# Autodesk Inventor assembly: Assembly1 DOLORIMETRO FINAL (ESPERO)
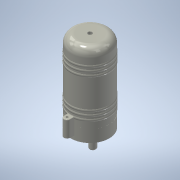
[picture p0: Inventor's stored thumbnail of the model, 180x180]
Saved by Autodesk Inventor 2022 (Build 260153000, 153)
## iProperties
Created: 2022-11-21
Part Number: Assembly1 DOLORIMETRO FINAL (ESPERO)
Document SubType Name: Assembly
Designer: ASUS
Author: ASUS
## Documents named in this file (5)
- C:\CICLO IV\FUNDAMENTOS DE BIODISEÑO\BIODEÑO\Assembly1 DOLORIMETRO FINAL (ESPERO).iam
- C:\CICLO IV\FUNDAMENTOS DE BIODISEÑO\BIODEÑO\BARRA V3 (1).ipt
- C:\CICLO IV\FUNDAMENTOS DE BIODISEÑO\BIODEÑO\Carcasa V3 (1)\Carcasa V3-01.ipt
- C:\CICLO IV\FUNDAMENTOS DE BIODISEÑO\BIODEÑO\Carcasa V3 (1).ipt
- C:\CICLO IV\FUNDAMENTOS DE BIODISEÑO\BIODEÑO\Carcasa V3 Pequeño (1).ipt
## Components (3 placed, 3 different names)
1. Carcasa V3-01:1 — Mate:1, Mate:4
2. Carcasa V3 Pequeño (1):1 — Mate:1, Mate:2, Mate:3, Mate:4
3. BARRA V3 (1):2 — Mate:2, Mate:3
## Relationships (4: Mate 4)
- Mate:1: Carcasa V3-01:1 ↔ Carcasa V3 Pequeño (1):1
- Mate:2: Carcasa V3 Pequeño (1):1 ↔ BARRA V3 (1):2
- Mate:3: Carcasa V3 Pequeño (1):1 ↔ BARRA V3 (1):2
- Mate:4: Carcasa V3-01:1 ↔ Carcasa V3 Pequeño (1):1
